# Autodesk Inventor assembly: winch
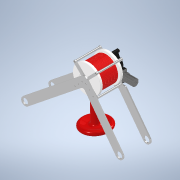
[picture p0: Inventor's stored thumbnail of the model, 180x180]
Saved by Autodesk Inventor 2020.2 (Build 242310000, 310)
## iProperties
Created: 2020-03-23
Part Number: winch
Document SubType Name: Assembly
Designer: agmle
Mass: 6591.71 g
Surface Area: 4788.14 cm^2
Volume: 2717.62 cm^3
Density: 2.42555 g/cm^3
Author: agmle
## Documents named in this file (17)
- D:\projects\CreekFleet_AutoBuoy\Mechanical CAD\station-keeping\winch.iam
- D:\projects\CreekFleet_AutoBuoy\Mechanical CAD\station-keeping\Window Motor Right.ipt
- D:\projects\CreekFleet_AutoBuoy\Mechanical CAD\station-keeping\winch_drum.ipt
- D:\projects\CreekFleet_AutoBuoy\Mechanical CAD\propulsion\bearing\6138k63.iam
- D:\projects\CreekFleet_AutoBuoy\Mechanical CAD\station-keeping\shaft.ipt
- D:\projects\CreekFleet_AutoBuoy\Mechanical CAD\station-keeping\motor_support.ipt
- \\rackstation\media\documents\Inventor\Content Center Files\R2020\en-US\ANSI B18.3.1M(6)\ANSI B18.3.1M - M5x0.8 x 40(1).ipt
- \\rackstation\media\documents\Inventor\Content Center Files\R2020\en-US\ANSI B18.3.1M(6)\ANSI B18.3.1M - M5x0.8 x 30(1).ipt
- D:\projects\CreekFleet_AutoBuoy\Mechanical CAD\station-keeping\strut.ipt
- \\rackstation\media\documents\Inventor\Content Center Files\R2020\en-US\ASME ANSI B18.3.5M(1)\ASME_ANSI B18.3.5M - M5x14(1).ipt
- D:\projects\CreekFleet_AutoBuoy\Mechanical CAD\station-keeping\winch_support.ipt
- D:\projects\CreekFleet_AutoBuoy\Mechanical CAD\station-keeping\anchor.ipt
- \\rackstation\media\documents\Inventor\Content Center Files\R2020\en-US\ANSI B18.22.1\ANSI B18.22.1 - No. 5 - narrow - Type B.ipt
- D:\projects\CreekFleet_AutoBuoy\Mechanical CAD\station-keeping\anchor_line.ipt
- D:\projects\CreekFleet_AutoBuoy\Mechanical CAD\station-keeping\winch_support_mount.ipt
- \\rackstation\media\documents\Inventor\Content Center Files\R2020\en-US\ASME ANSI B18.3.5M(1)\ASME_ANSI B18.3.5M - M3x10(1).ipt
- D:\projects\CreekFleet_AutoBuoy\Mechanical CAD\station-keeping\motor_support_mount.ipt
## Components (37 placed, 16 different names)
1. motor_support_mount:1 — Insert:35, Insert:36, Insert:37, Insert:38, Insert:39, Insert:40, Insert:41
2. Forged Hexagon Socket Flat Countersunk Head Cap Screws - Metric M3x10:7 — Insert:40
3. Forged Hexagon Socket Flat Countersunk Head Cap Screws - Metric M3x10:8 — Insert:41
4. Forged Hexagon Socket Flat Countersunk Head Cap Screws - Metric M3x10:9 — Insert:39
5. Forged Hexagon Socket Flat Countersunk Head Cap Screws - Metric M3x10:10 — Insert:38
6. Forged Hexagon Socket Flat Countersunk Head Cap Screws - Metric M3x10:11 — Insert:37
7. Plain Washer (Inch) No. 5 - narrow - Type B:1 — Insert:25, Insert:26
8. winch_drum:1 — Mate:1, Insert:25, Mate:2, Mate:5
9. 6138k63:1 [sub-assembly] — Insert:3, Insert:26, Insert:42
10. shaft:1 — Insert:3
11. Window Motor Right:1 — Mate:1, Insert:6, Insert:7, Insert:8, Insert:9, Insert:10
12. Forged Socket Head Cap Screw - Metric M5x0.8 x 40:1 — Insert:8
13. Forged Socket Head Cap Screw - Metric M5x0.8 x 30:1 — Insert:7
14. Forged Socket Head Cap Screw - Metric M5x0.8 x 30:2 — Insert:6
15. motor_support:1 — Insert:9, Insert:10, Insert:11, Insert:12, Insert:13, Insert:14, Insert:15, Insert:16, Insert:17, Insert:18, Insert:35, Insert:36
16. strut:1 — Insert:12, Insert:19
17. strut:2 — Insert:11, Insert:20
18. strut:3 — Insert:13
19. strut:4 — Insert:14
20. Forged Hexagon Socket Flat Countersunk Head Cap Screws - Metric M5x14:1 — Insert:15
21. Forged Hexagon Socket Flat Countersunk Head Cap Screws - Metric M5x14:2 — Insert:17
22. Forged Hexagon Socket Flat Countersunk Head Cap Screws - Metric M5x14:3 — Insert:16
23. Forged Hexagon Socket Flat Countersunk Head Cap Screws - Metric M5x14:4 — Insert:18
24. winch_support:1 — Insert:19, Insert:20, Insert:21, Insert:22, Insert:23, Insert:24, Insert:27, Insert:28, Insert:42
25. Forged Hexagon Socket Flat Countersunk Head Cap Screws - Metric M5x14:5 — Insert:24
26. Forged Hexagon Socket Flat Countersunk Head Cap Screws - Metric M5x14:6 — Insert:23
27. Forged Hexagon Socket Flat Countersunk Head Cap Screws - Metric M5x14:7 — Insert:22
28. Forged Hexagon Socket Flat Countersunk Head Cap Screws - Metric M5x14:8 — Insert:21
29. anchor:1 — Mate:3, Mate:4
30. anchor_line:1 — Mate:2, Mate:3, Mate:4, Mate:5
31. winch_support_mount:1 — Insert:27, Insert:28, Insert:29, Insert:30, Insert:31, Insert:32, Insert:33, Insert:34
32. Forged Hexagon Socket Flat Countersunk Head Cap Screws - Metric M3x10:1 — Insert:34
33. Forged Hexagon Socket Flat Countersunk Head Cap Screws - Metric M3x10:2 — Insert:33
34. Forged Hexagon Socket Flat Countersunk Head Cap Screws - Metric M3x10:3 — Insert:30
35. Forged Hexagon Socket Flat Countersunk Head Cap Screws - Metric M3x10:4 — Insert:29
36. Forged Hexagon Socket Flat Countersunk Head Cap Screws - Metric M3x10:5 — Insert:31
37. Forged Hexagon Socket Flat Countersunk Head Cap Screws - Metric M3x10:6 — Insert:32
## Relationships (43: Insert 38, Mate 5)
- Mate:1: winch_drum:1 ↔ Window Motor Right:1
- Insert:3: 6138k63:1 ↔ shaft:1
- Insert:6: Window Motor Right:1 ↔ Forged Socket Head Cap Screw - Metric M5x0.8 x 30:2
- Insert:7: Window Motor Right:1 ↔ Forged Socket Head Cap Screw - Metric M5x0.8 x 30:1
- Insert:8: Window Motor Right:1 ↔ Forged Socket Head Cap Screw - Metric M5x0.8 x 40:1
- Insert:9: Window Motor Right:1 ↔ motor_support:1
- Insert:10: Window Motor Right:1 ↔ motor_support:1
- Insert:11: motor_support:1 ↔ strut:2
- Insert:12: motor_support:1 ↔ strut:1
- Insert:13: motor_support:1 ↔ strut:3
- Insert:14: motor_support:1 ↔ strut:4
- Insert:15: motor_support:1 ↔ Forged Hexagon Socket Flat Countersunk Head Cap Screws - Metric M5x14:1
- Insert:16: motor_support:1 ↔ Forged Hexagon Socket Flat Countersunk Head Cap Screws - Metric M5x14:3
- Insert:17: motor_support:1 ↔ Forged Hexagon Socket Flat Countersunk Head Cap Screws - Metric M5x14:2
- Insert:18: motor_support:1 ↔ Forged Hexagon Socket Flat Countersunk Head Cap Screws - Metric M5x14:4
- Insert:19: strut:1 ↔ winch_support:1
- Insert:20: strut:2 ↔ winch_support:1
- Insert:21: winch_support:1 ↔ Forged Hexagon Socket Flat Countersunk Head Cap Screws - Metric M5x14:8
- Insert:22: winch_support:1 ↔ Forged Hexagon Socket Flat Countersunk Head Cap Screws - Metric M5x14:7
- Insert:23: winch_support:1 ↔ Forged Hexagon Socket Flat Countersunk Head Cap Screws - Metric M5x14:6
- Insert:24: winch_support:1 ↔ Forged Hexagon Socket Flat Countersunk Head Cap Screws - Metric M5x14:5
- Insert:25: Plain Washer (Inch) No. 5 - narrow - Type B:1 ↔ winch_drum:1
- Insert:26: Plain Washer (Inch) No. 5 - narrow - Type B:1 ↔ 6138k63:1
- Mate:2: winch_drum:1 ↔ anchor_line:1
- Mate:3: anchor:1 ↔ anchor_line:1
- Mate:4: anchor:1 ↔ anchor_line:1
- Mate:5: winch_drum:1 ↔ anchor_line:1
- Insert:27: winch_support:1 ↔ winch_support_mount:1
- Insert:28: winch_support:1 ↔ winch_support_mount:1
- Insert:29: winch_support_mount:1 ↔ Forged Hexagon Socket Flat Countersunk Head Cap Screws - Metric M3x10:4
- Insert:30: winch_support_mount:1 ↔ Forged Hexagon Socket Flat Countersunk Head Cap Screws - Metric M3x10:3
- Insert:31: winch_support_mount:1 ↔ Forged Hexagon Socket Flat Countersunk Head Cap Screws - Metric M3x10:5
- Insert:32: winch_support_mount:1 ↔ Forged Hexagon Socket Flat Countersunk Head Cap Screws - Metric M3x10:6
- Insert:33: winch_support_mount:1 ↔ Forged Hexagon Socket Flat Countersunk Head Cap Screws - Metric M3x10:2
- Insert:34: winch_support_mount:1 ↔ Forged Hexagon Socket Flat Countersunk Head Cap Screws - Metric M3x10:1
- Insert:35: motor_support_mount:1 ↔ motor_support:1
- Insert:36: motor_support_mount:1 ↔ motor_support:1
- Insert:37: motor_support_mount:1 ↔ Forged Hexagon Socket Flat Countersunk Head Cap Screws - Metric M3x10:11
- Insert:38: motor_support_mount:1 ↔ Forged Hexagon Socket Flat Countersunk Head Cap Screws - Metric M3x10:10
- Insert:39: motor_support_mount:1 ↔ Forged Hexagon Socket Flat Countersunk Head Cap Screws - Metric M3x10:9
- Insert:40: motor_support_mount:1 ↔ Forged Hexagon Socket Flat Countersunk Head Cap Screws - Metric M3x10:7
- Insert:41: motor_support_mount:1 ↔ Forged Hexagon Socket Flat Countersunk Head Cap Screws - Metric M3x10:8
- Insert:42: 6138k63:1 ↔ winch_support:1
